# Autodesk Inventor assembly: Foot
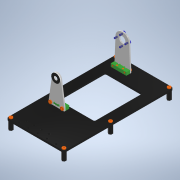
[picture p0: Inventor's stored thumbnail of the model, 180x180]
Saved by Autodesk Inventor 2020.4 (Build 244396000, 396)
## iProperties
Created: 2021-10-01
Part Number: Foot
Document SubType Name: Assembly
Designer: Masato Kubotera
Mass: 86.3924 g
Surface Area: 378.18 cm^2
Volume: 42.6269 cm^3
Density: 2.02671 g/cm^3
Author: Masato Kubotera
## Documents named in this file (10)
- C:\Users\Masato\Documents\Inventor\CIT Brains_Inventor\OpenPlatform_ver3_0 - ve4_1 branch\LowerBody\Foot\Foot.iam
- C:\Users\Masato\Documents\Inventor\CIT Brains_Inventor\OpenPlatform_ver3_0 - ve4_1 branch\LowerBody\Foot\Foot_back_frame.ipt
- C:\Users\Masato\Documents\Inventor\CIT Brains_Inventor\OpenPlatform_ver3_0 - ve4_1 branch\LowerBody\Foot\Foot_front_frame.ipt
- C:\Users\Masato\Documents\Inventor\CIT Brains_Inventor\OpenPlatform_ver3_0 - ve4_1 branch\LowerBody\Foot\Foot_root_block.ipt
- C:\Users\Masato\Documents\Inventor\CIT Brains_Inventor\OpenPlatform_ver3_0 - ve4_1 branch\LowerBody\Foot\Sole_frame.ipt
- C:\Users\Masato\Documents\Inventor\CIT Brains_Inventor\OpenPlatform_ver3_0 - ve4_1 branch\Ready_Made\Screw\M3-8.ipt
- C:\Users\Masato\Documents\Inventor\CIT Brains_Inventor\OpenPlatform_ver3_0 - ve4_1 branch\Ready_Made\Screw\M2_6-6.ipt
- C:\Users\Masato\Documents\Inventor\CIT Brains_Inventor\OpenPlatform_ver3_0 - ve4_1 branch\Ready_Made\TT-0814-10.ipt
- C:\Users\Masato\Documents\Inventor\CIT Brains_Inventor\OpenPlatform_ver3_0 - ve4_1 branch\Ready_Made\UUW-0614-05BH.ipt
- C:\Users\Masato\Documents\Inventor\CIT Brains_Inventor\OpenPlatform_ver3_0 - ve4_1 branch\Ready_Made\ASL-313BE.ipt
## Components (31 placed, 9 different names)
1. Foot_back_frame:1 — 挿入:11, 挿入:12, 挿入:35, 挿入:36, 挿入:37, 挿入:38, 挿入:43, 挿入:44
2. Foot_front_frame:1 — 挿入:13, 挿入:14, メイト:2, 挿入:39, 挿入:41, 挿入:42
3. Foot_root_block:1 — 挿入:7, 挿入:8, 挿入:13, 挿入:14
4. Foot_root_block:2 — 挿入:9, 挿入:10, 挿入:11, 挿入:12
5. Sole_frame:1 — メイト:1, フラッシュ:1, 挿入:7, 挿入:8, 挿入:9, 挿入:10, 挿入:17, 挿入:18, 挿入:19, 挿入:20, 挿入:21, 挿入:22, 挿入:27, 挿入:28, 挿入:29, 挿入:30, 挿入:45, 挿入:46, 挿入:47, 挿入:48, 挿入:49, 挿入:50
6. M3-8:1 — 挿入:17
7. M3-8:2 — 挿入:18
8. M3-8:3 — 挿入:19
9. M3-8:4 — 挿入:20
10. M3-8:5 — 挿入:21
11. M3-8:6 — 挿入:22
12. M3-8:7 — 挿入:27
13. M3-8:8 — 挿入:28
14. M3-8:9 — 挿入:29
15. M3-8:10 — 挿入:30
16. M2_6-6:1 — 挿入:35
17. M2_6-6:2 — 挿入:36
18. M2_6-6:3 — 挿入:37
19. M2_6-6:4 — 挿入:38
20. TT-0814-10:1 — 挿入:39, 挿入:40
21. UUW-0614-05BH:1 — 挿入:40
22. M3-8:11 — 挿入:42
23. M3-8:12 — 挿入:41
24. M3-8:13 — 挿入:43
25. M3-8:14 — 挿入:44
26. ASL-313BE:1 — 挿入:50
27. ASL-313BE:2 — 挿入:49
28. ASL-313BE:3 — 挿入:48
29. ASL-313BE:4 — 挿入:47
30. ASL-313BE:5 — 挿入:46
31. ASL-313BE:6 — 挿入:45
## Relationships (37: Insert 34, Mate 2, Flush 1)
- メイト:1 [Mate]: Sole_frame:1
- フラッシュ:1 [Flush]: Sole_frame:1
- 挿入:7 [Insert]: Foot_root_block:1 ↔ Sole_frame:1
- 挿入:8 [Insert]: Foot_root_block:1 ↔ Sole_frame:1
- 挿入:9 [Insert]: Foot_root_block:2 ↔ Sole_frame:1
- 挿入:10 [Insert]: Foot_root_block:2 ↔ Sole_frame:1
- 挿入:11 [Insert]: Foot_back_frame:1 ↔ Foot_root_block:2
- 挿入:12 [Insert]: Foot_back_frame:1 ↔ Foot_root_block:2
- 挿入:13 [Insert]: Foot_front_frame:1 ↔ Foot_root_block:1
- 挿入:14 [Insert]: Foot_front_frame:1 ↔ Foot_root_block:1
- 挿入:17 [Insert]: Sole_frame:1 ↔ M3-8:1
- 挿入:18 [Insert]: Sole_frame:1 ↔ M3-8:2
- 挿入:19 [Insert]: Sole_frame:1 ↔ M3-8:3
- 挿入:20 [Insert]: Sole_frame:1 ↔ M3-8:4
- 挿入:21 [Insert]: Sole_frame:1 ↔ M3-8:5
- 挿入:22 [Insert]: Sole_frame:1 ↔ M3-8:6
- メイト:2 [Mate]: Foot_front_frame:1
- 挿入:27 [Insert]: Sole_frame:1 ↔ M3-8:7
- 挿入:28 [Insert]: Sole_frame:1 ↔ M3-8:8
- 挿入:29 [Insert]: Sole_frame:1 ↔ M3-8:9
- 挿入:30 [Insert]: Sole_frame:1 ↔ M3-8:10
- 挿入:35 [Insert]: Foot_back_frame:1 ↔ M2_6-6:1
- 挿入:36 [Insert]: Foot_back_frame:1 ↔ M2_6-6:2
- 挿入:37 [Insert]: Foot_back_frame:1 ↔ M2_6-6:3
- 挿入:38 [Insert]: Foot_back_frame:1 ↔ M2_6-6:4
- 挿入:39 [Insert]: Foot_front_frame:1 ↔ TT-0814-10:1
- 挿入:40 [Insert]: TT-0814-10:1 ↔ UUW-0614-05BH:1
- 挿入:41 [Insert]: Foot_front_frame:1 ↔ M3-8:12
- 挿入:42 [Insert]: Foot_front_frame:1 ↔ M3-8:11
- 挿入:43 [Insert]: Foot_back_frame:1 ↔ M3-8:13
- 挿入:44 [Insert]: Foot_back_frame:1 ↔ M3-8:14
- 挿入:45 [Insert]: Sole_frame:1 ↔ ASL-313BE:6
- 挿入:46 [Insert]: Sole_frame:1 ↔ ASL-313BE:5
- 挿入:47 [Insert]: Sole_frame:1 ↔ ASL-313BE:4
- 挿入:48 [Insert]: Sole_frame:1 ↔ ASL-313BE:3
- 挿入:49 [Insert]: Sole_frame:1 ↔ ASL-313BE:2
- 挿入:50 [Insert]: Sole_frame:1 ↔ ASL-313BE:1
